# Autodesk Inventor assembly: HUB ASSEMBLY
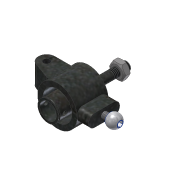
[picture p0: Inventor's stored thumbnail of the model, 180x180]
Saved by Autodesk Inventor 2016 (Build 200138000, 138)
## iProperties
Created: 2015-04-18
Part Number: HUB ASSEMBLY
Document SubType Name: Assembly
Designer: Station9
Author: Station9
## Documents named in this file (6)
- E:\worldskills Project\Project Archive\AD\AD-6(94.01.29)WSC2011\HUB ASSEMBLY.iam
- E:\worldskills Project\Project Archive\AD\AD-6(94.01.29)WSC2011\500-126.ipt
- E:\worldskills Project\Project Archive\AD\AD-6(94.01.29)WSC2011\500-007.ipt
- E:\worldskills Project\Project Archive\AD\AD-6(94.01.29)WSC2011\500-113.ipt
- E:\worldskills Project\Project Archive\AD\AD-6(94.01.29)WSC2011\Content Center\en-US\ISO 3245 (I)\ISO 3245 - 21 D - 10 x 14 x 7(1) I.ipt
- E:\worldskills Project\Project Archive\AD\AD-6(94.01.29)WSC2011\Content Center\en-US\ISO 4032(2)\ISO 4032 - M4ISO.ipt
## Components (5 placed, 5 different names)
1. 500-126:1 — Mate:1, Mate:7, Flush:1, Mate:9
2. 500-007:1 — Mate:1, Mate:4, Mate:6, Mate:8, Mate:9
3. 500-113:1 — Mate:4, Mate:6
4. ISO 3245 (I) 21 D - 10 x 14 x 7:1 — Mate:8
5. ISO 4032 M4:1 — Mate:7, Flush:1
## Relationships (7: Mate 6, Flush 1)
- Mate:1: 500-126:1 ↔ 500-007:1
- Mate:4: 500-007:1 ↔ 500-113:1
- Mate:6 (2.9 mm): 500-007:1 ↔ 500-113:1
- Mate:7: 500-126:1 ↔ ISO 4032 M4:1
- Flush:1 (1.6 mm): 500-126:1 ↔ ISO 4032 M4:1
- Mate:8: 500-007:1 ↔ ISO 3245 (I) 21 D - 10 x 14 x 7:1
- Mate:9: 500-126:1 ↔ 500-007:1
